# Autodesk Inventor assembly: hpc_Q2307-ACC
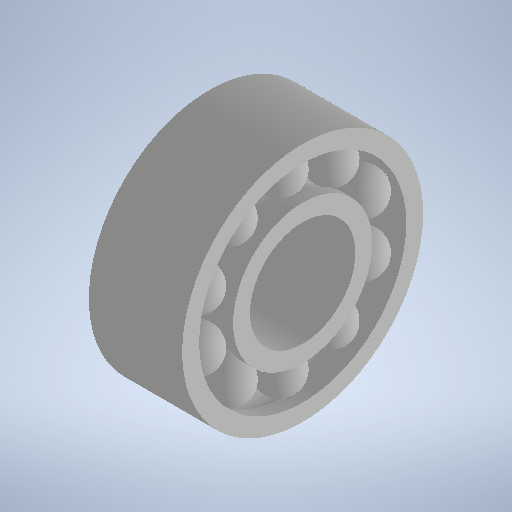
[picture p0: Inventor's stored thumbnail of the model, 512x512]
Saved by Autodesk Inventor 2025 (Build 290162000, 162)
## iProperties
Category: PARTsolutions
Company: HPC
Created: 2026-05-26
Part Number: hpc_Q2307-ACC
Catalog Web Link: www.3dfindit.com
Description: Q1Q2-Self-aligning radial ball bearing
Vendor: HPC
Document SubType Name: Assembly
Designer: psAdmin
Manufacturer: HPC
Mass: 680 g
Surface Area: 387.152 cm^2
Volume: 85.3514 cm^3
Density: 7.96706 g/cm^3
PSOL_IDENT_0: {$CADENAS_DATA/23d-libs/hpc/v3/rotary/radial/steel/q1q2.prj},181 {VTYP=3D},{STYP=ASSTAB},{NB=hpc_Q23
PSOL_IDENT_1: 07-ACC},{LINA=HPC - Q2307-ACC},{NN=Q1Q2},{DATE=17.02.2022 08:08:09},{GEOMDATE=12.01.2018 14:09:54},{
PSOL_IDENT_2: VERSION=},{LINEID=220},{WBVAR=},{WBNUMERIC=}  {NB=hpc_Q2307-ACC},{LINA=HPC - Q2307-ACC},{KT=DUMMY},{
PSOL_IDENT_3: REF=Q2307-ACC},{D=35},{D1=80},{B=31},{CD=38.91},{CS=10.98},{VLG=9180},{VLH=10800},{MAS=0.680},{INFO=
PSOL_IDENT_4: INFO},{PPATH=q1q2_asmtpl.prj},{HIDDENLINE=}
NB: hpc_Q2307-ACC
NN: Q1Q2
NT: Self-aligning radial ball bearing
NBSYN: hpc_$REF.
LINA: HPC - Q2307-ACC
CATALOG: HPC
REF: Q2307-ACC
D: 35
D1: 80
B: 31
CD: 38.91
CS: 10.98
VLG: 9180
VLH: 10800
MAS: 0.68
INFO: INFO
SUPPLIER: HPC
ARTICLENO: hpc_Q2307-ACC
BOMINFO: HPC - Q2307-ACC
CREATOR: CADENAS GmbH
Title: HPC - Q2307-ACC
Author: Cadenas PARTsolutions
Comments: Self-aligning radial ball bearing
## Documents named in this file (4)
- C:\Users\matot\OneDrive - Stellenbosch University\2026\MechatronicsProject478\Building the joint\Joint Assembly\hpc_Q2307-ACC.iam
- C:\Users\matot\OneDrive - Stellenbosch University\2026\MechatronicsProject478\Building the joint\Joint Assembly\hpc_Q2307-ACC_1.ipt
- C:\Users\matot\OneDrive - Stellenbosch University\2026\MechatronicsProject478\Building the joint\Joint Assembly\hpc_Q2307-ACC_2.ipt
- C:\Users\matot\OneDrive - Stellenbosch University\2026\MechatronicsProject478\Building the joint\Joint Assembly\hpc_Q2307-ACC_3.ipt
## Components (22 placed, 3 different names)
1. hpc_Q2307-ACC_1:1 — IP_2_XY@1 <-> IP_2_XY@2, IP_2_Z@1 <-> IP_2_Z@2, IP_2_YZ@1 <-> IP_2_YZ@2
2. hpc_Q2307-ACC_2:1 — IP_2_XY@1 <-> IP_2_XY@2, IP_2_Z@1 <-> IP_2_Z@2, IP_2_YZ@1 <-> IP_2_YZ@2, IP_3_1_XY@2 <-> IP_3_XY@3, IP_3_1_Z@2 <-> IP_3_Z@3, IP_3_1_YZ@2 <-> IP_3_YZ@3, IP_3_2_XY@2 <-> IP_3_XY@4, IP_3_2_Z@2 <-> IP_3_Z@4, IP_3_2_YZ@2 <-> IP_3_YZ@4, IP_3_3_XY@2 <-> IP_3_XY@5, IP_3_3_Z@2 <-> IP_3_Z@5, IP_3_3_YZ@2 <-> IP_3_YZ@5, IP_3_4_XY@2 <-> IP_3_XY@6, IP_3_4_Z@2 <-> IP_3_Z@6, IP_3_4_YZ@2 <-> IP_3_YZ@6, IP_3_5_XY@2 <-> IP_3_XY@7, IP_3_5_Z@2 <-> IP_3_Z@7, IP_3_5_YZ@2 <-> IP_3_YZ@7, IP_3_6_XY@2 <-> IP_3_XY@8, IP_3_6_Z@2 <-> IP_3_Z@8, IP_3_6_YZ@2 <-> IP_3_YZ@8, IP_3_7_XY@2 <-> IP_3_XY@9, IP_3_7_Z@2 <-> IP_3_Z@9, IP_3_7_YZ@2 <-> IP_3_YZ@9, IP_3_8_XY@2 <-> IP_3_XY@10, IP_3_8_Z@2 <-> IP_3_Z@10, IP_3_8_YZ@2 <-> IP_3_YZ@10, IP_3_9_XY@2 <-> IP_3_XY@11, IP_3_9_Z@2 <-> IP_3_Z@11, IP_3_9_YZ@2 <-> IP_3_YZ@11, IP_3_10_XY@2 <-> IP_3_XY@12, IP_3_10_Z@2 <-> IP_3_Z@12, IP_3_10_YZ@2 <-> IP_3_YZ@12, IP_4_1_XY@2 <-> IP_3_XY@13, IP_4_1_Z@2 <-> IP_3_Z@13, IP_4_1_YZ@2 <-> IP_3_YZ@13, IP_4_2_XY@2 <-> IP_3_XY@14, IP_4_2_Z@2 <-> IP_3_Z@14, IP_4_2_YZ@2 <-> IP_3_YZ@14, IP_4_3_XY@2 <-> IP_3_XY@15, IP_4_3_Z@2 <-> IP_3_Z@15, IP_4_3_YZ@2 <-> IP_3_YZ@15, IP_4_4_XY@2 <-> IP_3_XY@16, IP_4_4_Z@2 <-> IP_3_Z@16, IP_4_4_YZ@2 <-> IP_3_YZ@16, IP_4_5_XY@2 <-> IP_3_XY@17, IP_4_5_Z@2 <-> IP_3_Z@17, IP_4_5_YZ@2 <-> IP_3_YZ@17, IP_4_6_XY@2 <-> IP_3_XY@18, IP_4_6_Z@2 <-> IP_3_Z@18, IP_4_6_YZ@2 <-> IP_3_YZ@18, IP_4_7_XY@2 <-> IP_3_XY@19, IP_4_7_Z@2 <-> IP_3_Z@19, IP_4_7_YZ@2 <-> IP_3_YZ@19, IP_4_8_XY@2 <-> IP_3_XY@20, IP_4_8_Z@2 <-> IP_3_Z@20, IP_4_8_YZ@2 <-> IP_3_YZ@20, IP_4_9_XY@2 <-> IP_3_XY@21, IP_4_9_Z@2 <-> IP_3_Z@21, IP_4_9_YZ@2 <-> IP_3_YZ@21, IP_4_10_XY@2 <-> IP_3_XY@22, IP_4_10_Z@2 <-> IP_3_Z@22, IP_4_10_YZ@2 <-> IP_3_YZ@22
3. hpc_Q2307-ACC_3:1 — IP_3_1_XY@2 <-> IP_3_XY@3, IP_3_1_Z@2 <-> IP_3_Z@3, IP_3_1_YZ@2 <-> IP_3_YZ@3
4. hpc_Q2307-ACC_3:2 — IP_3_2_XY@2 <-> IP_3_XY@4, IP_3_2_Z@2 <-> IP_3_Z@4, IP_3_2_YZ@2 <-> IP_3_YZ@4
5. hpc_Q2307-ACC_3:3 — IP_3_3_XY@2 <-> IP_3_XY@5, IP_3_3_Z@2 <-> IP_3_Z@5, IP_3_3_YZ@2 <-> IP_3_YZ@5
6. hpc_Q2307-ACC_3:4 — IP_3_4_XY@2 <-> IP_3_XY@6, IP_3_4_Z@2 <-> IP_3_Z@6, IP_3_4_YZ@2 <-> IP_3_YZ@6
7. hpc_Q2307-ACC_3:5 — IP_3_5_XY@2 <-> IP_3_XY@7, IP_3_5_Z@2 <-> IP_3_Z@7, IP_3_5_YZ@2 <-> IP_3_YZ@7
8. hpc_Q2307-ACC_3:6 — IP_3_6_XY@2 <-> IP_3_XY@8, IP_3_6_Z@2 <-> IP_3_Z@8, IP_3_6_YZ@2 <-> IP_3_YZ@8
9. hpc_Q2307-ACC_3:7 — IP_3_7_XY@2 <-> IP_3_XY@9, IP_3_7_Z@2 <-> IP_3_Z@9, IP_3_7_YZ@2 <-> IP_3_YZ@9
10. hpc_Q2307-ACC_3:8 — IP_3_8_XY@2 <-> IP_3_XY@10, IP_3_8_Z@2 <-> IP_3_Z@10, IP_3_8_YZ@2 <-> IP_3_YZ@10
11. hpc_Q2307-ACC_3:9 — IP_3_9_XY@2 <-> IP_3_XY@11, IP_3_9_Z@2 <-> IP_3_Z@11, IP_3_9_YZ@2 <-> IP_3_YZ@11
12. hpc_Q2307-ACC_3:10 — IP_3_10_XY@2 <-> IP_3_XY@12, IP_3_10_Z@2 <-> IP_3_Z@12, IP_3_10_YZ@2 <-> IP_3_YZ@12
13. hpc_Q2307-ACC_3:11 — IP_4_1_XY@2 <-> IP_3_XY@13, IP_4_1_Z@2 <-> IP_3_Z@13, IP_4_1_YZ@2 <-> IP_3_YZ@13
14. hpc_Q2307-ACC_3:12 — IP_4_2_XY@2 <-> IP_3_XY@14, IP_4_2_Z@2 <-> IP_3_Z@14, IP_4_2_YZ@2 <-> IP_3_YZ@14
15. hpc_Q2307-ACC_3:13 — IP_4_3_XY@2 <-> IP_3_XY@15, IP_4_3_Z@2 <-> IP_3_Z@15, IP_4_3_YZ@2 <-> IP_3_YZ@15
16. hpc_Q2307-ACC_3:14 — IP_4_4_XY@2 <-> IP_3_XY@16, IP_4_4_Z@2 <-> IP_3_Z@16, IP_4_4_YZ@2 <-> IP_3_YZ@16
17. hpc_Q2307-ACC_3:15 — IP_4_5_XY@2 <-> IP_3_XY@17, IP_4_5_Z@2 <-> IP_3_Z@17, IP_4_5_YZ@2 <-> IP_3_YZ@17
18. hpc_Q2307-ACC_3:16 — IP_4_6_XY@2 <-> IP_3_XY@18, IP_4_6_Z@2 <-> IP_3_Z@18, IP_4_6_YZ@2 <-> IP_3_YZ@18
19. hpc_Q2307-ACC_3:17 — IP_4_7_XY@2 <-> IP_3_XY@19, IP_4_7_Z@2 <-> IP_3_Z@19, IP_4_7_YZ@2 <-> IP_3_YZ@19
20. hpc_Q2307-ACC_3:18 — IP_4_8_XY@2 <-> IP_3_XY@20, IP_4_8_Z@2 <-> IP_3_Z@20, IP_4_8_YZ@2 <-> IP_3_YZ@20
21. hpc_Q2307-ACC_3:19 — IP_4_9_XY@2 <-> IP_3_XY@21, IP_4_9_Z@2 <-> IP_3_Z@21, IP_4_9_YZ@2 <-> IP_3_YZ@21
22. hpc_Q2307-ACC_3:20 — IP_4_10_XY@2 <-> IP_3_XY@22, IP_4_10_Z@2 <-> IP_3_Z@22, IP_4_10_YZ@2 <-> IP_3_YZ@22
## Relationships (63: Flush 21, Mate 21, Angle 21)
- IP_2_XY@1 <-> IP_2_XY@2 [Flush]: hpc_Q2307-ACC_1:1 ↔ hpc_Q2307-ACC_2:1
- IP_2_Z@1 <-> IP_2_Z@2 [Mate]: hpc_Q2307-ACC_1:1 ↔ hpc_Q2307-ACC_2:1
- IP_2_YZ@1 <-> IP_2_YZ@2 [Angle] (0 deg): hpc_Q2307-ACC_1:1 ↔ hpc_Q2307-ACC_2:1
- IP_3_1_XY@2 <-> IP_3_XY@3 [Flush]: hpc_Q2307-ACC_2:1 ↔ hpc_Q2307-ACC_3:1
- IP_3_1_Z@2 <-> IP_3_Z@3 [Mate]: hpc_Q2307-ACC_2:1 ↔ hpc_Q2307-ACC_3:1
- IP_3_1_YZ@2 <-> IP_3_YZ@3 [Angle] (0 deg): hpc_Q2307-ACC_2:1 ↔ hpc_Q2307-ACC_3:1
- IP_3_2_XY@2 <-> IP_3_XY@4 [Flush]: hpc_Q2307-ACC_2:1 ↔ hpc_Q2307-ACC_3:2
- IP_3_2_Z@2 <-> IP_3_Z@4 [Mate]: hpc_Q2307-ACC_2:1 ↔ hpc_Q2307-ACC_3:2
- IP_3_2_YZ@2 <-> IP_3_YZ@4 [Angle] (0 deg): hpc_Q2307-ACC_2:1 ↔ hpc_Q2307-ACC_3:2
- IP_3_3_XY@2 <-> IP_3_XY@5 [Flush]: hpc_Q2307-ACC_2:1 ↔ hpc_Q2307-ACC_3:3
- IP_3_3_Z@2 <-> IP_3_Z@5 [Mate]: hpc_Q2307-ACC_2:1 ↔ hpc_Q2307-ACC_3:3
- IP_3_3_YZ@2 <-> IP_3_YZ@5 [Angle] (0 deg): hpc_Q2307-ACC_2:1 ↔ hpc_Q2307-ACC_3:3
- IP_3_4_XY@2 <-> IP_3_XY@6 [Flush]: hpc_Q2307-ACC_2:1 ↔ hpc_Q2307-ACC_3:4
- IP_3_4_Z@2 <-> IP_3_Z@6 [Mate]: hpc_Q2307-ACC_2:1 ↔ hpc_Q2307-ACC_3:4
- IP_3_4_YZ@2 <-> IP_3_YZ@6 [Angle] (0 deg): hpc_Q2307-ACC_2:1 ↔ hpc_Q2307-ACC_3:4
- IP_3_5_XY@2 <-> IP_3_XY@7 [Flush]: hpc_Q2307-ACC_2:1 ↔ hpc_Q2307-ACC_3:5
- IP_3_5_Z@2 <-> IP_3_Z@7 [Mate]: hpc_Q2307-ACC_2:1 ↔ hpc_Q2307-ACC_3:5
- IP_3_5_YZ@2 <-> IP_3_YZ@7 [Angle] (0 deg): hpc_Q2307-ACC_2:1 ↔ hpc_Q2307-ACC_3:5
- IP_3_6_XY@2 <-> IP_3_XY@8 [Flush]: hpc_Q2307-ACC_2:1 ↔ hpc_Q2307-ACC_3:6
- IP_3_6_Z@2 <-> IP_3_Z@8 [Mate]: hpc_Q2307-ACC_2:1 ↔ hpc_Q2307-ACC_3:6
- IP_3_6_YZ@2 <-> IP_3_YZ@8 [Angle] (0 deg): hpc_Q2307-ACC_2:1 ↔ hpc_Q2307-ACC_3:6
- IP_3_7_XY@2 <-> IP_3_XY@9 [Flush]: hpc_Q2307-ACC_2:1 ↔ hpc_Q2307-ACC_3:7
- IP_3_7_Z@2 <-> IP_3_Z@9 [Mate]: hpc_Q2307-ACC_2:1 ↔ hpc_Q2307-ACC_3:7
- IP_3_7_YZ@2 <-> IP_3_YZ@9 [Angle] (0 deg): hpc_Q2307-ACC_2:1 ↔ hpc_Q2307-ACC_3:7
- IP_3_8_XY@2 <-> IP_3_XY@10 [Flush]: hpc_Q2307-ACC_2:1 ↔ hpc_Q2307-ACC_3:8
- IP_3_8_Z@2 <-> IP_3_Z@10 [Mate]: hpc_Q2307-ACC_2:1 ↔ hpc_Q2307-ACC_3:8
- IP_3_8_YZ@2 <-> IP_3_YZ@10 [Angle] (0 deg): hpc_Q2307-ACC_2:1 ↔ hpc_Q2307-ACC_3:8
- IP_3_9_XY@2 <-> IP_3_XY@11 [Flush]: hpc_Q2307-ACC_2:1 ↔ hpc_Q2307-ACC_3:9
- IP_3_9_Z@2 <-> IP_3_Z@11 [Mate]: hpc_Q2307-ACC_2:1 ↔ hpc_Q2307-ACC_3:9
- IP_3_9_YZ@2 <-> IP_3_YZ@11 [Angle] (0 deg): hpc_Q2307-ACC_2:1 ↔ hpc_Q2307-ACC_3:9
- IP_3_10_XY@2 <-> IP_3_XY@12 [Flush]: hpc_Q2307-ACC_2:1 ↔ hpc_Q2307-ACC_3:10
- IP_3_10_Z@2 <-> IP_3_Z@12 [Mate]: hpc_Q2307-ACC_2:1 ↔ hpc_Q2307-ACC_3:10
- IP_3_10_YZ@2 <-> IP_3_YZ@12 [Angle] (0 deg): hpc_Q2307-ACC_2:1 ↔ hpc_Q2307-ACC_3:10
- IP_4_1_XY@2 <-> IP_3_XY@13 [Flush]: hpc_Q2307-ACC_2:1 ↔ hpc_Q2307-ACC_3:11
- IP_4_1_Z@2 <-> IP_3_Z@13 [Mate]: hpc_Q2307-ACC_2:1 ↔ hpc_Q2307-ACC_3:11
- IP_4_1_YZ@2 <-> IP_3_YZ@13 [Angle] (0 deg): hpc_Q2307-ACC_2:1 ↔ hpc_Q2307-ACC_3:11
- IP_4_2_XY@2 <-> IP_3_XY@14 [Flush]: hpc_Q2307-ACC_2:1 ↔ hpc_Q2307-ACC_3:12
- IP_4_2_Z@2 <-> IP_3_Z@14 [Mate]: hpc_Q2307-ACC_2:1 ↔ hpc_Q2307-ACC_3:12
- IP_4_2_YZ@2 <-> IP_3_YZ@14 [Angle] (0 deg): hpc_Q2307-ACC_2:1 ↔ hpc_Q2307-ACC_3:12
- IP_4_3_XY@2 <-> IP_3_XY@15 [Flush]: hpc_Q2307-ACC_2:1 ↔ hpc_Q2307-ACC_3:13
- IP_4_3_Z@2 <-> IP_3_Z@15 [Mate]: hpc_Q2307-ACC_2:1 ↔ hpc_Q2307-ACC_3:13
- IP_4_3_YZ@2 <-> IP_3_YZ@15 [Angle] (0 deg): hpc_Q2307-ACC_2:1 ↔ hpc_Q2307-ACC_3:13
- IP_4_4_XY@2 <-> IP_3_XY@16 [Flush]: hpc_Q2307-ACC_2:1 ↔ hpc_Q2307-ACC_3:14
- IP_4_4_Z@2 <-> IP_3_Z@16 [Mate]: hpc_Q2307-ACC_2:1 ↔ hpc_Q2307-ACC_3:14
- IP_4_4_YZ@2 <-> IP_3_YZ@16 [Angle] (0 deg): hpc_Q2307-ACC_2:1 ↔ hpc_Q2307-ACC_3:14
- IP_4_5_XY@2 <-> IP_3_XY@17 [Flush]: hpc_Q2307-ACC_2:1 ↔ hpc_Q2307-ACC_3:15
- IP_4_5_Z@2 <-> IP_3_Z@17 [Mate]: hpc_Q2307-ACC_2:1 ↔ hpc_Q2307-ACC_3:15
- IP_4_5_YZ@2 <-> IP_3_YZ@17 [Angle] (0 deg): hpc_Q2307-ACC_2:1 ↔ hpc_Q2307-ACC_3:15
- IP_4_6_XY@2 <-> IP_3_XY@18 [Flush]: hpc_Q2307-ACC_2:1 ↔ hpc_Q2307-ACC_3:16
- IP_4_6_Z@2 <-> IP_3_Z@18 [Mate]: hpc_Q2307-ACC_2:1 ↔ hpc_Q2307-ACC_3:16
- IP_4_6_YZ@2 <-> IP_3_YZ@18 [Angle] (0 deg): hpc_Q2307-ACC_2:1 ↔ hpc_Q2307-ACC_3:16
- IP_4_7_XY@2 <-> IP_3_XY@19 [Flush]: hpc_Q2307-ACC_2:1 ↔ hpc_Q2307-ACC_3:17
- IP_4_7_Z@2 <-> IP_3_Z@19 [Mate]: hpc_Q2307-ACC_2:1 ↔ hpc_Q2307-ACC_3:17
- IP_4_7_YZ@2 <-> IP_3_YZ@19 [Angle] (0 deg): hpc_Q2307-ACC_2:1 ↔ hpc_Q2307-ACC_3:17
- IP_4_8_XY@2 <-> IP_3_XY@20 [Flush]: hpc_Q2307-ACC_2:1 ↔ hpc_Q2307-ACC_3:18
- IP_4_8_Z@2 <-> IP_3_Z@20 [Mate]: hpc_Q2307-ACC_2:1 ↔ hpc_Q2307-ACC_3:18
- IP_4_8_YZ@2 <-> IP_3_YZ@20 [Angle] (0 deg): hpc_Q2307-ACC_2:1 ↔ hpc_Q2307-ACC_3:18
- IP_4_9_XY@2 <-> IP_3_XY@21 [Flush]: hpc_Q2307-ACC_2:1 ↔ hpc_Q2307-ACC_3:19
- IP_4_9_Z@2 <-> IP_3_Z@21 [Mate]: hpc_Q2307-ACC_2:1 ↔ hpc_Q2307-ACC_3:19
- IP_4_9_YZ@2 <-> IP_3_YZ@21 [Angle] (0 deg): hpc_Q2307-ACC_2:1 ↔ hpc_Q2307-ACC_3:19
- IP_4_10_XY@2 <-> IP_3_XY@22 [Flush]: hpc_Q2307-ACC_2:1 ↔ hpc_Q2307-ACC_3:20
- IP_4_10_Z@2 <-> IP_3_Z@22 [Mate]: hpc_Q2307-ACC_2:1 ↔ hpc_Q2307-ACC_3:20
- IP_4_10_YZ@2 <-> IP_3_YZ@22 [Angle] (0 deg): hpc_Q2307-ACC_2:1 ↔ hpc_Q2307-ACC_3:20
